# Autodesk Inventor assembly: 12TCircle
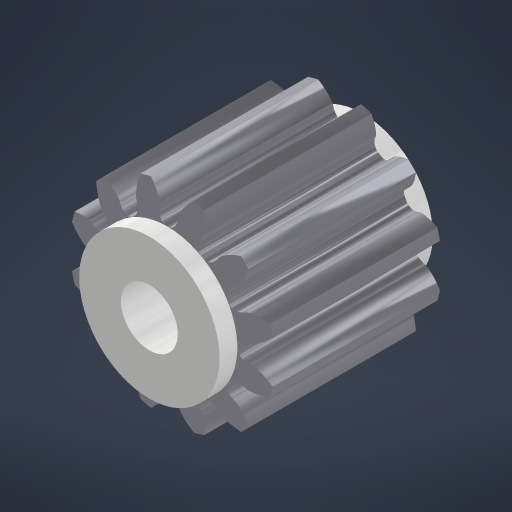
[picture p0: Inventor's stored thumbnail of the model, 512x512]
Saved by Autodesk Inventor 2023 (Build 270158000, 158)
## iProperties
Created: 2023-05-22
Part Number: 12TCircle
Document SubType Name: Assembly
Designer: alex
Author: alex
## Documents named in this file (4)
- C:\Users\alex\Documents\GitHub\4067X-Over-Under-CAD\Chassis\12TCircle.iam
- C:\Users\alex\Documents\GitHub\4067X-Over-Under-CAD\VEX-CAD-Inventor\Motion\Gears\HS Gear\HS 12T Gear, No Insert.iam
- C:\Users\alex\Documents\GitHub\4067X-Over-Under-CAD\VEX-CAD-Inventor\Motion\Gears\HS Gear.iam
- C:\Users\alex\Documents\GitHub\4067X-Over-Under-CAD\VEX-CAD-Inventor\Motion\Insert Circle.ipt
## Components (3 placed, 2 different names)
1. HS 12T Gear, No Insert:1 [sub-assembly] — Insert:1, Insert:2
2. Insert Circle:1 — Insert:1
3. Insert Circle:2 — Insert:2
## Relationships (2: Insert 2)
- Insert:1: HS 12T Gear, No Insert:1 ↔ Insert Circle:1
- Insert:2: HS 12T Gear, No Insert:1 ↔ Insert Circle:2
